# Autodesk Inventor assembly: ASY PRS 1200-80 top funnel
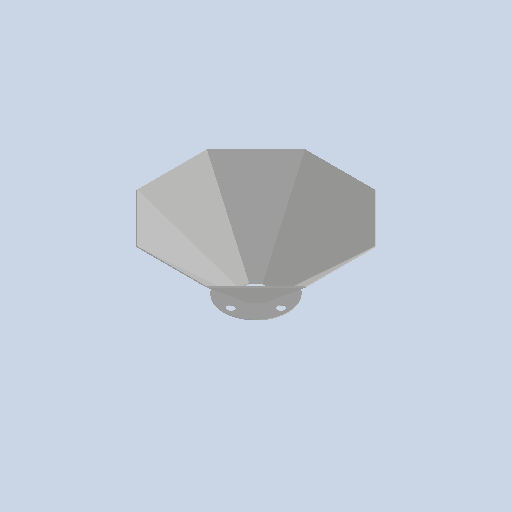
[picture p0: Inventor's stored thumbnail of the model, 512x512]
Saved by Autodesk Inventor 2025 (Build 290162010, 162A)
## iProperties
Created: 2025-07-11
Part Number: ASY PRS 1200-80 top funnel
Document SubType Name: Assembly
Designer: user
Mass: 3988.24 g
Surface Area: 4860.23 cm^2
Volume: 498.53 cm^3
Density: 8 g/cm^3
Author: user
## Documents named in this file (3)
- C:\Users\pokla\Documents\Inventor\PRS-Purovskii\Model\PRS-filter 1200\ASY PRS 1200-80 top funnel .iam
- C:\Users\pokla\Documents\Inventor\PRS-Purovskii\Model\PRS-filter 1200\PRS 1200-82 funnel FLANGE.ipt
- C:\Users\pokla\Documents\Inventor\PRS-Purovskii\Model\PRS-filter 1200\PRS 1200-81 top funnel.ipt
## Components (3 placed, 2 different names)
1. PRS 1200-82 funnel FLANGE.ipt:1 — Mate:2, Mate:1, Mate:4, Mate:3
2. PRS 1200-81 top funnel.ipt:1 — Mate:2, Mate:1, Mate:5
3. PRS 1200-81 top funnel.ipt:2 — Mate:5, Mate:4, Mate:3
## Relationships (5: Mate 5)
- Mate:2: PRS 1200-82 funnel FLANGE.ipt:1 ↔ PRS 1200-81 top funnel.ipt:1
- Mate:1: PRS 1200-82 funnel FLANGE.ipt:1 ↔ PRS 1200-81 top funnel.ipt:1
- Mate:5: PRS 1200-81 top funnel.ipt:1 ↔ PRS 1200-81 top funnel.ipt:2
- Mate:4: PRS 1200-82 funnel FLANGE.ipt:1 ↔ PRS 1200-81 top funnel.ipt:2
- Mate:3: PRS 1200-82 funnel FLANGE.ipt:1 ↔ PRS 1200-81 top funnel.ipt:2
